# Autodesk Inventor assembly: 202.001.01_Schieberbetaetigung
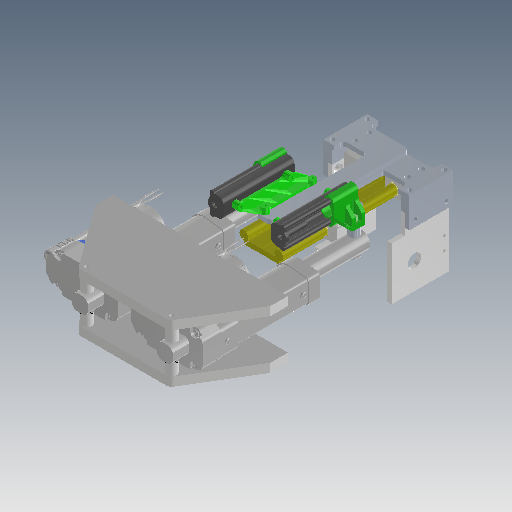
[picture p0: Inventor's stored thumbnail of the model, 512x512]
Saved by Autodesk Inventor 2021 (Build 250183000, 183)
## iProperties
Created: 2021-11-14
Part Number: 202.001.01_Schieberbetaetigung
Document SubType Name: Assembly
Designer: Oliver Ungerer
KODE_ZEICHNUNGSNUMMER: TFVEM_110M
BENENNUNG: Fuehrung Schieber
BEARBEITER_NAME: Ungerer O.
MASSE: 2.190774
PDMREV: 0.0+
PDMRL: Entwicklung
PROI_REVISION: 0
PROI_VERSION: 0+
PROI_RELEASE: Entwicklung
PTC_MODIFIED: True
PROI_CREATED_BY: Kantioler_adm
PROI_CREATED_ON: 07.03.2008 12:11:19
PROI_LOCATION: Root-Ordner/Pro_stds/Start_Files
MATERIALART: -
EINHEIT: ST
HERSTELLER_PREIS: 0.0
PRUEFER_NAME: Uo
PTC_ORGANIZATION_ID: Durst
PTC_WM_REVISION: 0
PTC_WM_ITERATION: 0
PTC_WM_VERSION: 0.0
PTC_WM_LIFECYCLE_STATE: Entwicklung
PTC_WM_LIFECYCLE: 02 Durst
PTC_WM_CREATED_BY: Oliver Ungerer (oungerer: Durst)
PTC_WM_CREATED_ON: 01.08.21
PTC_WM_MODIFIED_BY: Oliver Ungerer (oungerer: Durst)
PTC_WM_MODIFIED_ON: 01.08.21
AEND_INDEX: 0
VERSION: 0
STATUS: 0.0
Author: Oliver Ungerer
## Documents named in this file (20)
- \\u262868-sub23.your-storagebox.de@SSL\DavWWWRoot\Master_Projekt_SS_2021\Projektdaten\50_Modul_Vereinzelung\55_Konstruktion\102_Vereinzelung\202.001.01_Schieberbetaetigung.iam
- \\u262868-sub23.your-storagebox.de@SSL\DavWWWRoot\Master_Projekt_SS_2021\Projektdaten\50_Modul_Vereinzelung\55_Konstruktion\102_Vereinzelung\0001_IGUS_SCHIENE.ipt
- \\u262868-sub23.your-storagebox.de@SSL\DavWWWRoot\Master_Projekt_SS_2021\Projektdaten\50_Modul_Vereinzelung\55_Konstruktion\102_Vereinzelung\1346134.ipt
- \\u262868-sub23.your-storagebox.de@SSL\DavWWWRoot\Master_Projekt_SS_2021\Projektdaten\50_Modul_Vereinzelung\55_Konstruktion\102_Vereinzelung\TFVEM_10100.ipt
- \\u262868-sub23.your-storagebox.de@SSL\DavWWWRoot\Master_Projekt_SS_2021\Projektdaten\50_Modul_Vereinzelung\55_Konstruktion\102_Vereinzelung\TFVEM_1106.ipt
- \\u262868-sub23.your-storagebox.de@SSL\DavWWWRoot\Master_Projekt_SS_2021\Projektdaten\50_Modul_Vereinzelung\55_Konstruktion\102_Vereinzelung\TFVEM_1101.ipt
- \\u262868-sub23.your-storagebox.de@SSL\DavWWWRoot\Master_Projekt_SS_2021\Projektdaten\50_Modul_Vereinzelung\55_Konstruktion\102_Vereinzelung\TFVEM_10102.ipt
- \\u262868-sub23.your-storagebox.de@SSL\DavWWWRoot\Master_Projekt_SS_2021\Projektdaten\50_Modul_Vereinzelung\55_Konstruktion\102_Vereinzelung\TFVEM_10103.ipt
- \\u262868-sub23.your-storagebox.de@SSL\DavWWWRoot\Master_Projekt_SS_2021\Projektdaten\50_Modul_Vereinzelung\55_Konstruktion\102_Vereinzelung\TFVEM_10104.ipt
- \\u262868-sub23.your-storagebox.de@SSL\DavWWWRoot\Master_Projekt_SS_2021\Projektdaten\50_Modul_Vereinzelung\55_Konstruktion\102_Vereinzelung\202.001.02_Kraftlimitierung.iam
- \\u262868-sub23.your-storagebox.de@SSL\DavWWWRoot\Master_Projekt_SS_2021\Projektdaten\50_Modul_Vereinzelung\55_Konstruktion\102_Vereinzelung\202.001.03_Kraftlimitierung.iam
- \\u262868-sub23.your-storagebox.de@SSL\DavWWWRoot\Master_Projekt_SS_2021\Projektdaten\50_Modul_Vereinzelung\55_Konstruktion\102_Vereinzelung\CAHB-10-B1A-050158-AAAA0A-000.iam
- \\u262868-sub23.your-storagebox.de@SSL\DavWWWRoot\Master_Projekt_SS_2021\Projektdaten\50_Modul_Vereinzelung\55_Konstruktion\102_Vereinzelung\TFVEM_10105.ipt
- \\u262868-sub23.your-storagebox.de@SSL\DavWWWRoot\Master_Projekt_SS_2021\Projektdaten\50_Modul_Vereinzelung\55_Konstruktion\102_Vereinzelung\TFVEM_1009.ipt
- \\u262868-sub23.your-storagebox.de@SSL\DavWWWRoot\Master_Projekt_SS_2021\Projektdaten\50_Modul_Vereinzelung\55_Konstruktion\102_Vereinzelung\1237347.ipt
- \\u262868-sub23.your-storagebox.de@SSL\DavWWWRoot\Master_Projekt_SS_2021\Projektdaten\50_Modul_Vereinzelung\55_Konstruktion\102_Vereinzelung\1126405.ipt
- \\u262868-sub23.your-storagebox.de@SSL\DavWWWRoot\Master_Projekt_SS_2021\Projektdaten\50_Modul_Vereinzelung\55_Konstruktion\102_Vereinzelung\1126767.ipt
- \\u262868-sub23.your-storagebox.de@SSL\DavWWWRoot\Master_Projekt_SS_2021\Projektdaten\50_Modul_Vereinzelung\55_Konstruktion\102_Vereinzelung\202.001.04_Zapfen_Aktor.ipt
- \\u262868-sub23.your-storagebox.de@SSL\DavWWWRoot\Master_Projekt_SS_2021\Projektdaten\50_Modul_Vereinzelung\55_Konstruktion\102_Vereinzelung\202.001.05_Zapfen_Aktor_Auflage.ipt
- \\u262868-sub23.your-storagebox.de@SSL\DavWWWRoot\Master_Projekt_SS_2021\Projektdaten\50_Modul_Vereinzelung\55_Konstruktion\102_Vereinzelung\202.001.05_Anbindung_Aktor.ipt
## Components (31 placed, 20 different names)
1. 0001_IGUS_SCHIENE
2. 1346134
3. 1346134:1
4. 1346134:2
5. 1346134:3
6. TFVEM_10100
7. TFVEM_1106
8. TFVEM_1101
9. TFVEM_10100:1
10. TFVEM_10102
11. TFVEM_10103
12. TFVEM_10102:1
13. TFVEM_10104
14. 202.001.02_Kraftlimitierung [sub-assembly]
15. 202.001.03_Kraftlimitierung [sub-assembly]
16. 502.001.01_Linearaktor [sub-assembly] — Passend:1, Passend:2
17. CAHB-10-B1A-050158-AAAA0A-000:1 [sub-assembly] — Passend:3, Passend:4
18. TFVEM_10105
19. TFVEM_1009
20. 1237347
21. 1237347:1
22. 1126405
23. 1126405:1
24. 1126767
25. 1126767:1
26. 202.001.04_Zapfen_Aktor:1 — Passend:3, Passend:4, Passend:7, Passend:8
27. 202.001.04_Zapfen_Aktor:2 — Passend:1, Passend:2, Passend:5, Passend:6
28. 202.001.05_Zapfen_Aktor_Auflage:3 — Passend:7, Passend:8
29. 202.001.05_Zapfen_Aktor_Auflage:4 — Passend:5, Passend:6
30. 202.001.05_Anbindung_Aktor:1
31. 202.001.05_Anbindung_Aktor:2
## Relationships (14: Mate 14)
- Passend:1 [Mate] (1 mm): 502.001.01_Linearaktor ↔ 202.001.04_Zapfen_Aktor:2
- Passend:2 [Mate]: 502.001.01_Linearaktor ↔ 202.001.04_Zapfen_Aktor:2
- Passend:3 [Mate] (1 mm): CAHB-10-B1A-050158-AAAA0A-000:1 ↔ 202.001.04_Zapfen_Aktor:1
- Passend:4 [Mate]: CAHB-10-B1A-050158-AAAA0A-000:1 ↔ 202.001.04_Zapfen_Aktor:1
- Passend:5 [Mate]: 202.001.04_Zapfen_Aktor:2 ↔ 202.001.05_Zapfen_Aktor_Auflage:4
- Passend:6 [Mate]: 202.001.04_Zapfen_Aktor:2 ↔ 202.001.05_Zapfen_Aktor_Auflage:4
- Passend:7 [Mate]: 202.001.04_Zapfen_Aktor:1 ↔ 202.001.05_Zapfen_Aktor_Auflage:3
- Passend:8 [Mate]: 202.001.04_Zapfen_Aktor:1 ↔ 202.001.05_Zapfen_Aktor_Auflage:3
- [Mate]: 202.001.04_Zapfen_Aktor:2 ↔ 202.001.05_Anbindung_Aktor:1
- [Mate]: 202.001.04_Zapfen_Aktor:2 ↔ 202.001.05_Anbindung_Aktor:1
- [Mate]: 202.001.04_Zapfen_Aktor:1 ↔ 202.001.05_Anbindung_Aktor:1
- [Mate]: 202.001.05_Zapfen_Aktor_Auflage:4 ↔ 202.001.05_Anbindung_Aktor:2
- [Mate]: 202.001.05_Zapfen_Aktor_Auflage:3 ↔ 202.001.05_Anbindung_Aktor:2
- [Mate]: 202.001.05_Zapfen_Aktor_Auflage:4 ↔ 202.001.05_Anbindung_Aktor:2
## Named parameters: d8_d2 = 0 mm, d9_d3 = 0 mm, d10_d4 = 0 mm, d11_d6 = 0 mm, d12_d7 = 0 mm
